# Autodesk Inventor assembly: Wing Left
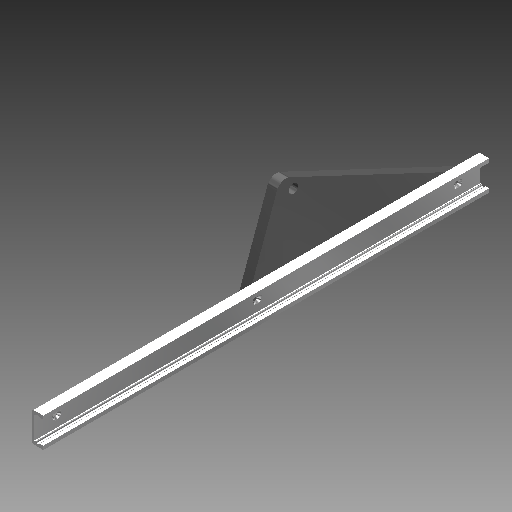
[picture p0: Inventor's stored thumbnail of the model, 512x512]
Saved by Autodesk Inventor 2019 (Build 230136000, 136)
## iProperties
Part Number: Wing Left
Document SubType Name: Assembly
Designer: Delta
Author: Delta
## Documents named in this file (3)
- C:\Robotics\2019-20_CAD\Collection\Wing Left.iam
- C:\Robotics\2019-20_CAD\Collection\Triangle axle slide connector.ipt
- C:\Robotics\COTSParts\Misumi_Slides\AIS2018\SAR330-30_b.ipt
## Components (2 placed, 2 different names)
1. Triangle axle slide connector:1 — Flush:1, Mate:1, Flush:2, Mate:2
2. SAR330-30_b:1 — Flush:1, Mate:1, Flush:2, Mate:2
## Relationships (4: Flush 2, Mate 2)
- Flush:1: Triangle axle slide connector:1 ↔ SAR330-30_b:1
- Mate:1: Triangle axle slide connector:1 ↔ SAR330-30_b:1
- Flush:2 (139.954 mm): Triangle axle slide connector:1 ↔ SAR330-30_b:1
- Mate:2 (0.01 mm): Triangle axle slide connector:1 ↔ SAR330-30_b:1
